# Autodesk Inventor assembly: sestava_SERVO
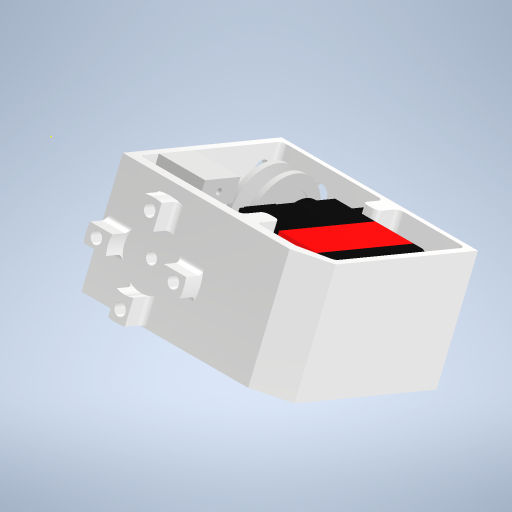
[picture p0: Inventor's stored thumbnail of the model, 512x512]
Saved by Autodesk Inventor 2023.1 (Build 271208000, 208)
## iProperties
Created: 2023-01-06
Part Number: sestava_SERVO
Document SubType Name: Assembly
Designer: zavrel
Author: zavrel
## Documents named in this file (9)
- C:\Users\zavrel\Documents\_OWNCLOUD_ACTUAL_WORK\GACR_Tensegrity\35_pohon_pro_Miletin\sestava_pohonu_SERVO\sestava_SERVO.iam
- C:\Users\zavrel\Documents\_OWNCLOUD_ACTUAL_WORK\GACR_Tensegrity\35_pohon_pro_Miletin\sestava_pohonu_SERVO\telo_pohonu.ipt
- C:\Users\zavrel\Documents\_OWNCLOUD_ACTUAL_WORK\GACR_Tensegrity\35_pohon_pro_Miletin\sestava_pohonu_SERVO\SERVO_PDI_6221MG.ipt
- C:\Users\zavrel\Documents\_OWNCLOUD_ACTUAL_WORK\GACR_Tensegrity\35_pohon_pro_Miletin\sestava_pohonu_SERVO\bubinek_sestava.iam
- C:\Users\zavrel\Documents\_OWNCLOUD_ACTUAL_WORK\GACR_Tensegrity\35_pohon_pro_Miletin\sestava_pohonu_SERVO\talirek_servo.ipt
- C:\Users\zavrel\Documents\_OWNCLOUD_ACTUAL_WORK\GACR_Tensegrity\35_pohon_pro_Miletin\sestava_pohonu_SERVO\drzak_pritlaku.ipt
- C:\Users\zavrel\Documents\_OWNCLOUD_ACTUAL_WORK\GACR_Tensegrity\35_pohon_pro_Miletin\sestava_pohonu_SERVO\drzak_pritlacneho_kolecka.ipt
- C:\Users\zavrel\Documents\_OWNCLOUD_ACTUAL_WORK\GACR_Tensegrity\35_pohon_pro_Miletin\sestava_pohonu_SERVO\uchyceni_pruziny.ipt
- C:\Users\zavrel\Documents\_OWNCLOUD_ACTUAL_WORK\GACR_Tensegrity\35_pohon_pro_Miletin\sestava_pohonu_SERVO\pritlacne_kolecko_sestava.iam
## Components (8 placed, 8 different names)
1. SERVO_PDI_6221MG:1 — Rigid:4, Rigid:2
2. telo_pohonu:1 — Rigid:4, Rigid:3, Tuhé:5
3. bubinek_sestava:1 [sub-assembly] — Rigid:1
4. talirek_servo:1 — Rigid:1, Rigid:2
5. drzak_pritlaku:1 — Rigid:3, Rotational:3
6. drzak_pritlacneho_kolecka:1 — Rotational:3, Rotational:4
7. uchyceni_pruziny:1 — Tuhé:5
8. pritlacne_kolecko_sestava:1 [sub-assembly] — Rotational:4
## Relationships (7: WeldJoint 5, RevoluteJoint 2)
- Rigid:4 [WeldJoint]: SERVO_PDI_6221MG:1 ↔ telo_pohonu:1
- Rigid:1 [WeldJoint]: bubinek_sestava:1 ↔ talirek_servo:1
- Rigid:2 [WeldJoint]: SERVO_PDI_6221MG:1 ↔ talirek_servo:1
- Rigid:3 [WeldJoint]: telo_pohonu:1 ↔ drzak_pritlaku:1
- Rotational:3 [RevoluteJoint] (0.25 mm): drzak_pritlaku:1 ↔ drzak_pritlacneho_kolecka:1
- Tuhé:5 [WeldJoint]: telo_pohonu:1 ↔ uchyceni_pruziny:1
- Rotational:4 [RevoluteJoint] (-0.25 mm): drzak_pritlacneho_kolecka:1 ↔ pritlacne_kolecko_sestava:1
